# Autodesk Inventor assembly: flexipod_v2_simplified_assembly
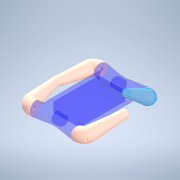
[picture p0: Inventor's stored thumbnail of the model, 180x180]
Saved by Autodesk Inventor 2020.2 (Build 242310000, 310)
## iProperties
Created: 2020-09-26
Part Number: flexipod_v2_simplified_assembly
Document SubType Name: Assembly
Designer: boxi
Author: boxi
## Documents named in this file (3)
- C:\Users\boxi\Documents\flexipod_hardware\mechanical_model\flexipod_assembly_simplified.iam
- C:\Users\boxi\Documents\flexipod_hardware\mechanical_model\soft_body_simplified.ipt
- C:\Users\boxi\Documents\flexipod_hardware\mechanical_model\leg.ipt
## Components (5 placed, 2 different names)
1. soft_body_simplified:1 — Rotational:1, Rotational:2, Rotational:3, Rotational:4
2. leg:1 — Rotational:1
3. leg:2 — Rotational:2
4. leg:3 — Rotational:3
5. leg:4 — Rotational:4
## Relationships (4: RevoluteJoint 4)
- Rotational:1 [RevoluteJoint] (2.2 mm): soft_body_simplified:1 ↔ leg:1
- Rotational:2 [RevoluteJoint] (2.2 mm): soft_body_simplified:1 ↔ leg:2
- Rotational:3 [RevoluteJoint] (2.2 mm): soft_body_simplified:1 ↔ leg:3
- Rotational:4 [RevoluteJoint] (2.2 mm): soft_body_simplified:1 ↔ leg:4
## Named parameters: leg_coupler_thickness = 2.2 mm
